# Autodesk Inventor assembly: MechanicalPalm
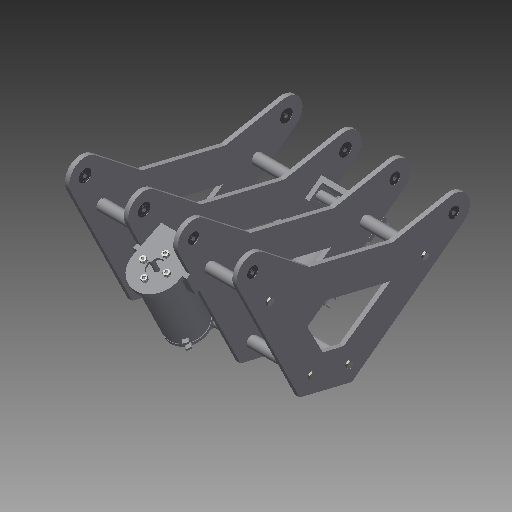
[picture p0: Inventor's stored thumbnail of the model, 512x512]
Saved by Autodesk Inventor 2018 (Build 220112000, 112)
## iProperties
Created: 2017-06-01
Part Number: MechanicalPalm
Document SubType Name: Weldment
Designer: Damian
Weld Material: Welded Aluminum-6061
Author: Damian
## Documents named in this file (10)
- C:\Users\Damian\MechanicalHand\CAD\MechanicalPalm.iam
- C:\Users\Damian\MechanicalHand\CAD\BaseCenterPlate.ipt
- C:\Users\Damian\MechanicalHand\CAD\BaseJointMotorMount.ipt
- C:\Users\Damian\MechanicalHand\StandardParts\3564_B\3564_B.ipt
- C:\Users\Damian\MechanicalHand\StandardParts\Bearing\Bearing.ipt
- C:\Users\Damian\MechanicalHand\CAD\BushingSmall.ipt
- C:\Users\Damian\Documents\Inventor\Content Center Files\R2018\en-US\AS 1420\AS 1420 - 1973 - M3 x 6.ipt
- C:\Users\Damian\MechanicalHand\CAD\BushingLarge.ipt
- C:\Users\Damian\MechanicalHand\CAD\BushingLargest.ipt
- C:\Users\Damian\Documents\Inventor\Content Center Files\R2018\en-US\AS 1110\AS 1110 - M3 x 6.ipt
## Components (44 placed, 9 different names)
1. BaseCenterPlate:1 — Mate:1, Mate:2, Mate:3, Mate:4, Mate:5, Mate:6, Mate:18, Mate:21, Mate:22, Mate:24, Mate:25, Mate:31, Mate:33, Mate:47, Mate:49
2. BaseCenterPlate:2 — Mate:7, Mate:8, Mate:9, Mate:16, Mate:19, Mate:20, Mate:23, Mate:30, Mate:38, Mate:46
3. BaseJointMotorMount:1 — Mate:4, Mate:5, Mate:6, Mate:7, Mate:8, Mate:9, Mate:10, Mate:11, Mate:12, Mate:26, Mate:27, Insert:1
4. BaseJointMotorMount:2 — Mate:1, Mate:2, Mate:3, Mate:13, Mate:14, Mate:15, Mate:28, Mate:29, Insert:2
5. 3564_B:1 — Mate:10, Mate:11, Mate:12
6. 3564_B:2 — Mate:13, Mate:14, Mate:15
7. Bearing:1 — Mate:19, Mate:23, Mate:36
8. Bearing:2 — Mate:18, Mate:24, Mate:25, Mate:35
9. Bearing:3 — Mate:21, Mate:22, Mate:34
10. Bearing:4 — Mate:16, Mate:20, Mate:37
11. BushingSmall:1 — Mate:28, Mate:29
12. BushingSmall:2 — Mate:26, Mate:27
13. BushingLarge:1 — Mate:33, Mate:47
14. BushingLarge:2 — Mate:30, Mate:31
15. BaseCenterPlate:3 — Mate:36, Mate:37, Mate:39, Mate:40, Mate:41, Mate:42, Mate:43, Mate:44, Mate:45, Mate:59, Mate:60, Mate:63, Mate:64, Insert:3, Insert:4, Insert:5, Insert:6
16. BaseCenterPlate:4 — Mate:34, Mate:35, Mate:48, Mate:50, Mate:51, Mate:52, Mate:53, Mate:54, Mate:55, Mate:56, Mate:57, Mate:58, Mate:61, Mate:62, Insert:7, Insert:8, Insert:9, Insert:10
17. BushingLargest:1 — Mate:53, Mate:54
18. BushingLargest:2 — Mate:48, Mate:49, Mate:50
19. BushingLargest:3 — Mate:38, Mate:39
20. BushingLargest:4 — Mate:43, Mate:44
21. BushingLargest:5 — Mate:42, Mate:45, Mate:46
22. BushingLargest:6 — Mate:40, Mate:41
23. BushingLargest:7 — Mate:55, Mate:56
24. BushingLargest:8 — Mate:51, Mate:52
25. Bearing:5 — Mate:59, Mate:63
26. Bearing:6 — Mate:60, Mate:64
27. Bearing:7 — Mate:57, Mate:61
28. Bearing:8 — Mate:58, Mate:62
29. AS 1110 - Metric M3 x 6:1 — Insert:3
30. AS 1110 - Metric M3 x 6:2 — Insert:4
31. AS 1110 - Metric M3 x 6:3 — Insert:5
32. AS 1110 - Metric M3 x 6:4 — Insert:6
33. AS 1110 - Metric M3 x 6:5 — Insert:7
34. AS 1110 - Metric M3 x 6:6 — Insert:8
35. AS 1110 - Metric M3 x 6:7 — Insert:9
36. AS 1110 - Metric M3 x 6:8 — Insert:10
37. AS 1420 - Metric M3 x 6:1 — Insert:1
38. AS 1420 - Metric M3 x 6:2
39. AS 1420 - Metric M3 x 6:3
40. AS 1420 - Metric M3 x 6:4
41. AS 1420 - Metric M3 x 6:5 — Insert:2
42. AS 1420 - Metric M3 x 6:6
43. AS 1420 - Metric M3 x 6:7
44. AS 1420 - Metric M3 x 6:8
## Component patterns: (4 elements, first: AS 1420 - Metric M3 x 6:1), (4 elements, first: AS 1420 - Metric M3 x 6:5)
## Relationships (72: Mate 62, Insert 10)
- Mate:1: BaseCenterPlate:1 ↔ BaseJointMotorMount:2
- Mate:2: BaseCenterPlate:1 ↔ BaseJointMotorMount:2
- Mate:3: BaseCenterPlate:1 ↔ BaseJointMotorMount:2
- Mate:4: BaseCenterPlate:1 ↔ BaseJointMotorMount:1
- Mate:5: BaseCenterPlate:1 ↔ BaseJointMotorMount:1
- Mate:6: BaseCenterPlate:1 ↔ BaseJointMotorMount:1
- Mate:7: BaseCenterPlate:2 ↔ BaseJointMotorMount:1
- Mate:8: BaseCenterPlate:2 ↔ BaseJointMotorMount:1
- Mate:9: BaseCenterPlate:2 ↔ BaseJointMotorMount:1
- Mate:10: BaseJointMotorMount:1 ↔ 3564_B:1
- Mate:11: BaseJointMotorMount:1 ↔ 3564_B:1
- Mate:12: BaseJointMotorMount:1 ↔ 3564_B:1
- Mate:13: BaseJointMotorMount:2 ↔ 3564_B:2
- Mate:14: BaseJointMotorMount:2 ↔ 3564_B:2
- Mate:15: BaseJointMotorMount:2 ↔ 3564_B:2
- Mate:16: BaseCenterPlate:2 ↔ Bearing:4
- Mate:18: BaseCenterPlate:1 ↔ Bearing:2
- Mate:19: BaseCenterPlate:2 ↔ Bearing:1
- Mate:20: BaseCenterPlate:2 ↔ Bearing:4
- Mate:21: BaseCenterPlate:1 ↔ Bearing:3
- Mate:22: BaseCenterPlate:1 ↔ Bearing:3
- Mate:23: BaseCenterPlate:2 ↔ Bearing:1
- Mate:24: BaseCenterPlate:1 ↔ Bearing:2
- Mate:25: BaseCenterPlate:1 ↔ Bearing:2
- Mate:26: BaseJointMotorMount:1 ↔ BushingSmall:2
- Mate:27: BaseJointMotorMount:1 ↔ BushingSmall:2
- Mate:28: BaseJointMotorMount:2 ↔ BushingSmall:1
- Mate:29: BaseJointMotorMount:2 ↔ BushingSmall:1
- Insert:1: BaseJointMotorMount:1 ↔ AS 1420 - Metric M3 x 6:1
- Insert:2: BaseJointMotorMount:2 ↔ AS 1420 - Metric M3 x 6:5
- Mate:30: BaseCenterPlate:2 ↔ BushingLarge:2
- Mate:31: BaseCenterPlate:1 ↔ BushingLarge:2
- Mate:33: BaseCenterPlate:1 ↔ BushingLarge:1
- Mate:34: Bearing:3 ↔ BaseCenterPlate:4
- Mate:35: Bearing:2 ↔ BaseCenterPlate:4
- Mate:36: Bearing:1 ↔ BaseCenterPlate:3
- Mate:37: Bearing:4 ↔ BaseCenterPlate:3
- Mate:38: BaseCenterPlate:2 ↔ BushingLargest:3
- Mate:39: BaseCenterPlate:3 ↔ BushingLargest:3
- Mate:40: BaseCenterPlate:3 ↔ BushingLargest:6
- Mate:41: BaseCenterPlate:3 ↔ BushingLargest:6
- Mate:42: BaseCenterPlate:3 ↔ BushingLargest:5
- Mate:43: BaseCenterPlate:3 ↔ BushingLargest:4
- Mate:44: BaseCenterPlate:3 ↔ BushingLargest:4
- Mate:45: BaseCenterPlate:3 ↔ BushingLargest:5
- Mate:46: BaseCenterPlate:2 ↔ BushingLargest:5
- Mate:47: BaseCenterPlate:1 ↔ BushingLarge:1
- Mate:48: BaseCenterPlate:4 ↔ BushingLargest:2
- Mate:49: BaseCenterPlate:1 ↔ BushingLargest:2
- Mate:50: BaseCenterPlate:4 ↔ BushingLargest:2
- Mate:51: BaseCenterPlate:4 ↔ BushingLargest:8
- Mate:52: BaseCenterPlate:4 ↔ BushingLargest:8
- Mate:53: BaseCenterPlate:4 ↔ BushingLargest:1
- Mate:54: BaseCenterPlate:4 ↔ BushingLargest:1
- Mate:55: BaseCenterPlate:4 ↔ BushingLargest:7
- Mate:56: BaseCenterPlate:4 ↔ BushingLargest:7
- Mate:57: BaseCenterPlate:4 ↔ Bearing:7
- Mate:58: BaseCenterPlate:4 ↔ Bearing:8
- Mate:59: BaseCenterPlate:3 ↔ Bearing:5
- Mate:60: BaseCenterPlate:3 ↔ Bearing:6
- Mate:61: BaseCenterPlate:4 ↔ Bearing:7
- Mate:62: BaseCenterPlate:4 ↔ Bearing:8
- Mate:63: BaseCenterPlate:3 ↔ Bearing:5
- Mate:64: BaseCenterPlate:3 ↔ Bearing:6
- Insert:3: BaseCenterPlate:3 ↔ AS 1110 - Metric M3 x 6:1
- Insert:4: BaseCenterPlate:3 ↔ AS 1110 - Metric M3 x 6:2
- Insert:5: BaseCenterPlate:3 ↔ AS 1110 - Metric M3 x 6:3
- Insert:6: BaseCenterPlate:3 ↔ AS 1110 - Metric M3 x 6:4
- Insert:7: BaseCenterPlate:4 ↔ AS 1110 - Metric M3 x 6:5
- Insert:8: BaseCenterPlate:4 ↔ AS 1110 - Metric M3 x 6:6
- Insert:9: BaseCenterPlate:4 ↔ AS 1110 - Metric M3 x 6:7
- Insert:10: BaseCenterPlate:4 ↔ AS 1110 - Metric M3 x 6:8
